# Autodesk Inventor assembly: Hudson 1-60.ipt
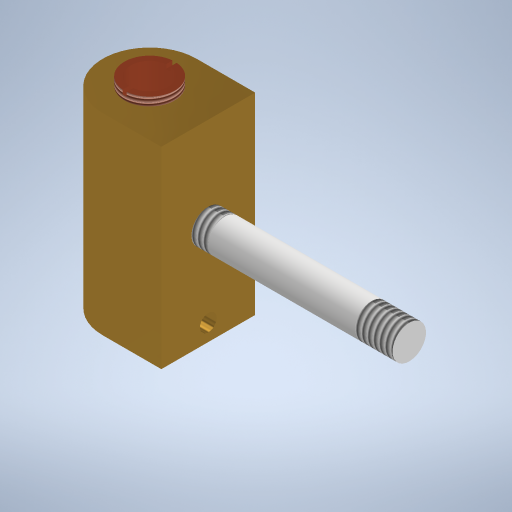
[picture p0: Inventor's stored thumbnail of the model, 512x512]
Saved by Autodesk Inventor 2024.2 (Build 282272000, 272)
## iProperties
Created: 2024-11-02
Part Number: Hudson 1-60.ipt
Document SubType Name: Assembly
Designer: Monica Mora
Author: Monica Mora
## Documents named in this file (6)
- C:\Users\Monica Mora\Desktop\Proyecto Locomotora\Hudson 1-60.ipt.iam
- C:\Users\Monica Mora\Desktop\Proyecto Locomotora\Pieza 1 subesnamble 1-60.ipt
- C:\Users\Monica Mora\Desktop\Proyecto Locomotora\Pieza 2 subensamble 1-60.ipt
- C:\Users\Monica Mora\Desktop\Proyecto Locomotora\Pieza 3 subensamble 1-60.ipt
- C:\Users\Monica Mora\Desktop\Proyecto Locomotora\Pieza 4 subensamble 1-60.ipt
- C:\Users\Monica Mora\Desktop\Proyecto Locomotora\Pieza 5 subensamble 1-60.ipt
## Components (5 placed, 5 different names)
1. Pieza 1 subesnamble 1-60:1 — Coincidencia:1, Coincidencia:2, Coincidencia:3, Coincidencia:5, Coincidencia:6, Coincidencia:7, Coincidencia:8
2. Pieza 2 subensamble 1-60:1 — Coincidencia:1, Coincidencia:2, Coincidencia:4
3. Pieza 3 subensamble 1-60:1 — Coincidencia:3, Coincidencia:4
4. Pieza 4 subensamble 1-60:1 — Coincidencia:5, Coincidencia:6
5. Pieza 5 subensamble 1-60:1 — Coincidencia:7, Coincidencia:8
## Relationships (8: Mate 8)
- Coincidencia:1 [Mate]: Pieza 1 subesnamble 1-60:1 ↔ Pieza 2 subensamble 1-60:1
- Coincidencia:2 [Mate]: Pieza 1 subesnamble 1-60:1 ↔ Pieza 2 subensamble 1-60:1
- Coincidencia:3 [Mate]: Pieza 1 subesnamble 1-60:1 ↔ Pieza 3 subensamble 1-60:1
- Coincidencia:4 [Mate]: Pieza 2 subensamble 1-60:1 ↔ Pieza 3 subensamble 1-60:1
- Coincidencia:5 [Mate]: Pieza 1 subesnamble 1-60:1 ↔ Pieza 4 subensamble 1-60:1
- Coincidencia:6 [Mate]: Pieza 1 subesnamble 1-60:1 ↔ Pieza 4 subensamble 1-60:1
- Coincidencia:7 [Mate]: Pieza 1 subesnamble 1-60:1 ↔ Pieza 5 subensamble 1-60:1
- Coincidencia:8 [Mate]: Pieza 1 subesnamble 1-60:1 ↔ Pieza 5 subensamble 1-60:1
